# Autodesk Inventor assembly: !flywheel
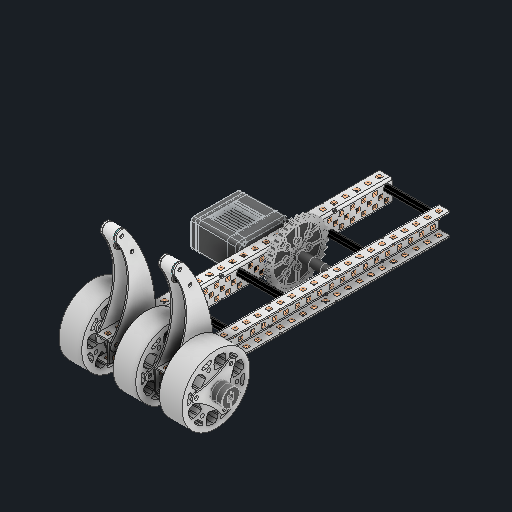
[picture p0: Inventor's stored thumbnail of the model, 512x512]
Saved by Autodesk Inventor 2024 (Build 280153000, 153)
## iProperties
Created: 2023-11-20
Part Number: !flywheel
Document SubType Name: Assembly
Designer: avere
Author: avere
## Documents named in this file (24)
- C:\Users\avere\Documents\rbp_cad\zoomba_v0.1\flywheel\!flywheel.iam
- C:\Users\avere\Documents\rbp_cad\VEX-CAD-Inventor-1.41\Structure\C Channel\Aluminum 1x2x1\Alu C 1x2x1x25.ipt
- C:\Users\avere\Documents\rbp_cad\VEX-CAD-Inventor-1.41\Structure\Standoff\Standoff 2.00.ipt
- C:\Users\avere\Documents\rbp_cad\VEX-CAD-Inventor-1.41\Structure\Standoff.ipt
- C:\Users\avere\Documents\rbp_cad\VEX-CAD-Inventor-1.41\Electronics\Motors with Screws\SteelM-StarS.iam
- C:\Users\avere\Documents\rbp_cad\VEX-CAD-Inventor-1.41\Electronics\Motors with Screws.iam
- C:\Users\avere\Documents\rbp_cad\VEX-CAD-Inventor-1.41\Motion\Wheels\Flex Wheels\3.000 Flex Wheel\3.000 30A 1.000.ipt
- C:\Users\avere\Documents\rbp_cad\VEX-CAD-Inventor-1.41\Motion\Wheels\Flex Wheels\3.000 Flex Wheel.ipt
- C:\Users\avere\Documents\rbp_cad\zoomba_v0.1\custom_parts\flex_wheel_hub.ipt
- C:\Users\avere\Documents\rbp_cad\VEX-CAD-Inventor-1.41\Motion\Wheels\Flex Wheels\VersaHex Adapters .125.ipt
- C:\Users\avere\Documents\rbp_cad\VEX-CAD-Inventor-1.41\Motion\Sprockets\6P Sprocket\6P 32T Sprocket, No Insert.iam
- C:\Users\avere\Documents\rbp_cad\VEX-CAD-Inventor-1.41\Motion\Sprockets\6P Sprocket.iam
- C:\Users\avere\Documents\rbp_cad\VEX-CAD-Inventor-1.41\Motion\Sprockets\6P Sprocket\6P 8T Sprocket, No Insert.iam
- C:\Users\avere\Documents\rbp_cad\VEX-CAD-Inventor-1.41\Motion\Spacers\Spacer Nylon .375 OD\NSpacer .375 OD x .500.ipt
- C:\Users\avere\Documents\rbp_cad\VEX-CAD-Inventor-1.41\Motion\Spacers\Spacer Nylon .375 OD.ipt
- C:\Users\avere\Documents\rbp_cad\VEX-CAD-Inventor-1.41\Motion\Shaft HS\HS Shaft Collar.ipt
- C:\Users\avere\Documents\rbp_cad\zoomba_v0.1\flywheel\custom_parts\triball_jig.ipt
- C:\Users\avere\Documents\rbp_cad\VEX-CAD-Inventor-1.41\Motion\Spacers\Spacer Nylon .500 OD\NSpacer White .500 OD x .500.ipt
- C:\Users\avere\Documents\rbp_cad\VEX-CAD-Inventor-1.41\Motion\Spacers\Spacer Nylon .500 OD.ipt
- C:\Users\avere\Documents\rbp_cad\zoomba_v0.1\chassis\custom_parts\thin_wide_washer.ipt
- C:\Users\avere\Documents\rbp_cad\VEX-CAD-Inventor-1.41\Motion\Spacers\Washer Steel\SWasher .375 OD x .015625.ipt
- C:\Users\avere\Documents\rbp_cad\VEX-CAD-Inventor-1.41\Motion\Spacers\Washer Steel.ipt
- C:\Users\avere\Documents\rbp_cad\VEX-CAD-Inventor-1.41\Motion\Spacers\Washer Steel\SWasher .375 OD x .062500.ipt
- C:\Users\avere\Documents\rbp_cad\VEX-CAD-Inventor-1.41\Structure\Standoff\Standoff .50.ipt
## Components (43 placed, 16 different names)
1. Alu C 1x2x1x25:1 — Insert:1, Insert:4, Insert:5, Insert:19, Insert:21, Insert:22, Mate:9, Insert:23, Insert:28, Insert:31, Insert:45, Mate:14
2. Alu C 1x2x1x25:2 — Insert:1, Insert:20, Mate:10, Insert:44, Mate:13
3. Standoff 2.00:1 — Insert:28, Mate:10
4. Standoff 2.00:3 — Insert:4
5. Standoff 2.00:4 — Insert:5
6. SteelM-StarS:1 [sub-assembly] — Insert:22, Mate:9
7. 3.000 30A 1.000:1 — Insert:7, Mate:3, Insert:8, Insert:10, Mate:4
8. flex_wheel_hub:1 — Insert:7, Mate:3
9. flex_wheel_hub:2 — Insert:9, Insert:10, Mate:4
10. VersaHex Adapters .125:1 — Insert:8, Insert:19, Insert:24
11. VersaHex Adapters .125:2 — Insert:9
12. 3.000 30A 1.000:2
13. flex_wheel_hub:3
14. flex_wheel_hub:4
15. VersaHex Adapters .125:3 — Insert:20
16. VersaHex Adapters .125:4 — Insert:29
17. 3.000 30A 1.000:3
18. flex_wheel_hub:5
19. flex_wheel_hub:6
20. VersaHex Adapters .125:5 — Insert:21
21. VersaHex Adapters .125:6 — Insert:30
22. 6P 32T Sprocket, No Insert:1 [sub-assembly] — Insert:23, Insert:27
23. 6P 8T Sprocket, No Insert:2 [sub-assembly] — Insert:24
24. NSpacer .375 OD x .500:1 — Insert:25
25. NSpacer .375 OD x .500:2 — Insert:25, Insert:26
26. NSpacer .375 OD x .500:3 — Insert:26, Insert:27
27. HS Shaft Collar:1 — Insert:29
28. HS Shaft Collar:2 — Insert:30
29. Standoff 2.00:5 — Insert:31
30. triball_jig:1 — Insert:37, Mate:11, Mate:13
31. triball_jig:2 — Insert:34, Insert:36, Insert:44
32. NSpacer White .500 OD x .500:1 — Insert:32, Mate:11
33. thin_wide_washer:1 — Insert:32, Insert:33
34. SWasher .375 OD x .015625:1 — Insert:33, Insert:34
35. SWasher .375 OD x .062500:2 — Insert:35, Insert:37
36. Standoff .50:6 — Insert:35, Insert:36
37. triball_jig:3
38. triball_jig:4 — Insert:45, Mate:14
39. NSpacer White .500 OD x .500:2
40. thin_wide_washer:2
41. SWasher .375 OD x .015625:3
42. SWasher .375 OD x .062500:4
43. Standoff .50:7
## Relationships (54: Insert 42, Mate 12)
- Insert:1 (50.8 mm): Alu C 1x2x1x25:1 ↔ Alu C 1x2x1x25:2
- Insert:4: Alu C 1x2x1x25:1 ↔ Standoff 2.00:3
- Insert:5: Alu C 1x2x1x25:1 ↔ Standoff 2.00:4
- Insert:7: 3.000 30A 1.000:1 ↔ flex_wheel_hub:1
- Mate:3: 3.000 30A 1.000:1 ↔ flex_wheel_hub:1
- Insert:8 (1.5875 mm): 3.000 30A 1.000:1 ↔ VersaHex Adapters .125:1
- Insert:9: flex_wheel_hub:2 ↔ VersaHex Adapters .125:2
- Insert:10: 3.000 30A 1.000:1 ↔ flex_wheel_hub:2
- Mate:4: 3.000 30A 1.000:1 ↔ flex_wheel_hub:2
- [Insert]: 3.000 30A 1.000:2 ↔ flex_wheel_hub:3
- [Mate]: 3.000 30A 1.000:2 ↔ flex_wheel_hub:3
- [Insert] (1.5875 mm): 3.000 30A 1.000:2 ↔ VersaHex Adapters .125:3
- [Insert]: flex_wheel_hub:4 ↔ VersaHex Adapters .125:4
- [Insert]: 3.000 30A 1.000:2 ↔ flex_wheel_hub:4
- [Mate]: 3.000 30A 1.000:2 ↔ flex_wheel_hub:4
- [Insert]: 3.000 30A 1.000:3 ↔ flex_wheel_hub:5
- [Mate]: 3.000 30A 1.000:3 ↔ flex_wheel_hub:5
- [Insert] (1.5875 mm): 3.000 30A 1.000:3 ↔ VersaHex Adapters .125:5
- [Insert]: flex_wheel_hub:6 ↔ VersaHex Adapters .125:6
- [Insert]: 3.000 30A 1.000:3 ↔ flex_wheel_hub:6
- [Mate]: 3.000 30A 1.000:3 ↔ flex_wheel_hub:6
- Insert:19 (13.0969 mm): Alu C 1x2x1x25:1 ↔ VersaHex Adapters .125:1
- Insert:20 (12.7 mm): Alu C 1x2x1x25:2 ↔ VersaHex Adapters .125:3
- Insert:21 (12.7 mm): Alu C 1x2x1x25:1 ↔ VersaHex Adapters .125:5
- Insert:22: Alu C 1x2x1x25:1 ↔ SteelM-StarS:1
- Mate:9: Alu C 1x2x1x25:1 ↔ SteelM-StarS:1
- Insert:23: Alu C 1x2x1x25:1 ↔ 6P 32T Sprocket, No Insert:1
- Insert:24: VersaHex Adapters .125:1 ↔ 6P 8T Sprocket, No Insert:2
- Insert:25: NSpacer .375 OD x .500:1 ↔ NSpacer .375 OD x .500:2
- Insert:26: NSpacer .375 OD x .500:2 ↔ NSpacer .375 OD x .500:3
- Insert:27: 6P 32T Sprocket, No Insert:1 ↔ NSpacer .375 OD x .500:3
- Insert:28: Alu C 1x2x1x25:1 ↔ Standoff 2.00:1
- Mate:10: Alu C 1x2x1x25:2 ↔ Standoff 2.00:1
- Insert:29: VersaHex Adapters .125:4 ↔ HS Shaft Collar:1
- Insert:30: VersaHex Adapters .125:6 ↔ HS Shaft Collar:2
- Insert:31: Alu C 1x2x1x25:1 ↔ Standoff 2.00:5
- Insert:32: NSpacer White .500 OD x .500:1 ↔ thin_wide_washer:1
- Insert:33: thin_wide_washer:1 ↔ SWasher .375 OD x .015625:1
- Insert:34: triball_jig:2 ↔ SWasher .375 OD x .015625:1
- Insert:35: SWasher .375 OD x .062500:2 ↔ Standoff .50:6
- Insert:36: triball_jig:2 ↔ Standoff .50:6
- Insert:37: triball_jig:1 ↔ SWasher .375 OD x .062500:2
- Mate:11: triball_jig:1 ↔ NSpacer White .500 OD x .500:1
- [Insert]: NSpacer White .500 OD x .500:2 ↔ thin_wide_washer:2
- [Insert]: thin_wide_washer:2 ↔ SWasher .375 OD x .015625:3
- [Insert]: triball_jig:4 ↔ SWasher .375 OD x .015625:3
- [Insert]: SWasher .375 OD x .062500:4 ↔ Standoff .50:7
- [Insert]: triball_jig:4 ↔ Standoff .50:7
- [Insert]: triball_jig:3 ↔ SWasher .375 OD x .062500:4
- [Mate]: triball_jig:3 ↔ NSpacer White .500 OD x .500:2
- Insert:44 (12.7 mm): Alu C 1x2x1x25:2 ↔ triball_jig:2
- Mate:13: Alu C 1x2x1x25:2 ↔ triball_jig:1
- Insert:45: Alu C 1x2x1x25:1 ↔ triball_jig:4
- Mate:14: Alu C 1x2x1x25:1 ↔ triball_jig:4
## Named parameters: d14_d8 = 0 mm, d15_d9 = 0 mm, d16_d10 = 1.5875 mm, d17_d11 = 0 mm, d18_d12 = 0 mm, d19_d13 = 0 mm, d20_d8 = 0 mm, d21_d9 = 0 mm, d22_d10 = 1.5875 mm, d23_d11 = 0 mm, d24_d12 = 0 mm, d25_d13 = 0 mm, d50_d43 = 0 mm, d51_d44 = 0 mm, d52_d45 = 0 mm, d53_d46 = 0 mm, d54_d47 = 0 mm, d55_d48 = 0 mm, d56_d49 = 0 mm
